# Autodesk Inventor assembly: Assembly 2017_08_31
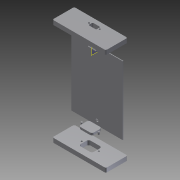
[picture p0: Inventor's stored thumbnail of the model, 180x180]
Saved by Autodesk Inventor 2012 (Build 160160000, 160)
## iProperties
Created: 2017-04-26
Part Number: Assembly 2017_08_31
Document SubType Name: Assembly
Designer: Brandon
Author: Brandon
## Documents named in this file (6)
- C:\Users\Brandon\Dropbox\Admiral Instruments Dropbox\power supply\power supply enclosure rev 2\Assembly 2017_08_31.iam
- C:\Users\Brandon\Dropbox\Admiral Instruments Dropbox\power supply\power supply enclosure rev 2\PCB.ipt
- C:\Users\Brandon\Dropbox\Admiral Instruments Dropbox\power supply\power supply enclosure rev 2\back cover.ipt
- C:\Users\Brandon\Dropbox\Admiral Instruments Dropbox\power supply\power supply enclosure rev 2\front cover.ipt
- C:\Users\Brandon\Dropbox\Admiral Instruments Dropbox\power supply\power supply enclosure rev 2\DB9 connector 2017_06_14.ipt
- C:\Users\Brandon\Dropbox\Admiral Instruments Dropbox\power supply\power supply enclosure rev 2\AC entry module.ipt
## Components (5 placed, 5 different names)
1. PCB:1 — Flush:5, Insert:10, Angle:9, Insert:11
2. back cover:1 — Mate:3, Mate:4, Flush:4, Flush:5
3. front cover:1 — Flush:3, Mate:2, Flush:4, Angle:10
4. DB9 connector 2017_06_14:1 — Insert:10, Angle:9
5. AC entry module:1 — Insert:11, Angle:10
## Relationships (10: Flush 3, Mate 3, Insert 2, Angle 2)
- Flush:3 (114.3 mm): front cover:1
- Mate:2: front cover:1
- Mate:3 (114.3 mm): back cover:1
- Mate:4: back cover:1
- Flush:4: back cover:1 ↔ front cover:1
- Flush:5 (7.2898 mm): PCB:1 ↔ back cover:1
- Insert:10: PCB:1 ↔ DB9 connector 2017_06_14:1
- Angle:9 (0 deg): PCB:1 ↔ DB9 connector 2017_06_14:1
- Insert:11: PCB:1 ↔ AC entry module:1
- Angle:10 (0 deg): front cover:1 ↔ AC entry module:1
